# Autodesk Inventor assembly: all_body
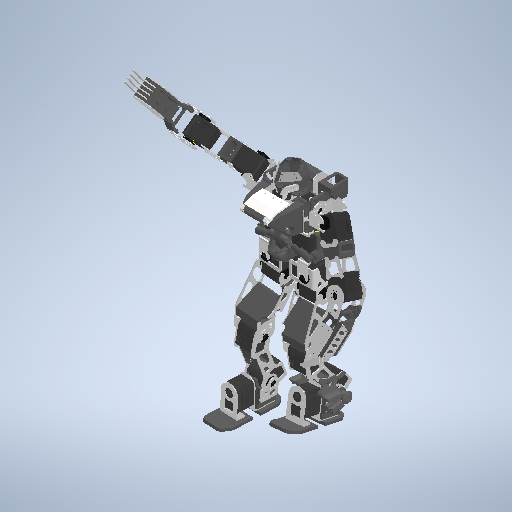
[picture p0: Inventor's stored thumbnail of the model, 512x512]
Saved by Autodesk Inventor 2026.1 (Build 301233020, 233B)
## iProperties
Created: 2024-10-10
Part Number: all_body
Document SubType Name: Assembly
Designer: hibik
Author: hibik
## Documents named in this file (5)
- C:\Users\hibik\Documents\Robomech\HR\Eglantyne_mark2\hard\all_body.iam
- C:\Users\hibik\Documents\Robomech\HR\Eglantyne_mark2\hard\body.iam
- C:\Users\hibik\Documents\Robomech\HR\Eglantyne_mark2\hard\leg\leg_right.iam
- C:\Users\hibik\Documents\Robomech\HR\Eglantyne_mark2\hard\leg\leg_left.iam
- C:\Users\hibik\Documents\Robomech\HR\Eglantyne_mark2\hard\arm\arm.iam
## Components (5 placed, 4 different names)
1. body:1 [sub-assembly] — 挿入:1, 挿入:2, 挿入:3, 挿入:4
2. leg_right:1 [sub-assembly] — 挿入:1
3. leg_left:1 [sub-assembly] — 挿入:2
4. arm:3 [sub-assembly] — 挿入:4
5. arm:4 [sub-assembly] — 挿入:3
## Relationships (4: Insert 4)
- 挿入:1 [Insert]: body:1 ↔ leg_right:1
- 挿入:2 [Insert]: body:1 ↔ leg_left:1
- 挿入:3 [Insert]: body:1 ↔ arm:4
- 挿入:4 [Insert]: body:1 ↔ arm:3
